# Autodesk Inventor assembly: XY Joint-Unit [A]
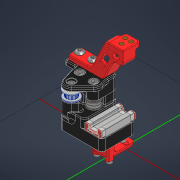
[picture p0: Inventor's stored thumbnail of the model, 180x180]
Saved by Autodesk Inventor 2022.2 (Build 262287010, 287A)
## iProperties
Created: 2022-03-15
Part Number: XY Joint-Unit [A]
Document SubType Name: Assembly
Designer: sleib
Author: sleib
## Documents named in this file (15)
- C:\Users\sleib\Projekte\Voron-2\CAD\Inventor\XY Joint-Unit [A].iam
- C:\Users\sleib\Projekte\Voron-2\CAD\Inventor\MGN9H Carriage.ipt
- C:\Users\sleib\Projekte\Voron-2\CAD\Inventor\M3x16 SHCS.ipt
- C:\Users\sleib\Projekte\Voron-2\CAD\Inventor\M3x30 SHCS.ipt
- C:\Users\sleib\Projekte\Voron-2\CAD\Inventor\XY Endstop Mount (Omron).ipt
- C:\Users\sleib\Projekte\Voron-2\CAD\Inventor\M5x40 SHCS.ipt
- C:\Users\sleib\Projekte\Voron-2\CAD\Inventor\GT2 20T Idler (6mm).ipt
- C:\Users\sleib\Projekte\Voron-2\CAD\Inventor\M5 Hexnut.ipt
- C:\Users\sleib\Projekte\Voron-2\CAD\Inventor\M5 Spacer (1mm).ipt
- C:\Users\sleib\Projekte\Voron-2\CAD\Inventor\Bearing F695-ZZ.ipt
- C:\Users\sleib\Projekte\Voron-2\CAD\Inventor\Chain Standoff (3-Hole).ipt
- C:\Users\sleib\Projekte\Voron-2\CAD\Inventor\M5x16 BHCS.ipt
- C:\Users\sleib\Projekte\Voron-2\CAD\Inventor\M5x30 BHCS.ipt
- C:\Users\sleib\Projekte\Voron-2\CAD\Inventor\XY Joint MGN12H [A].ipt
- C:\Users\sleib\Projekte\Voron-2\CAD\Inventor\M3 Threaded Insert.ipt
## Components (26 placed, 14 different names)
1. XY Joint MGN12H [A]:1 — Passend:50, Passend:51, Passend:52, Passend:53, Passend:54, Passend:55, Passend:56, Passend:57, Winkel:1, Winkel:2, Winkel:3, Passend:58, Passend:59, Passend:60, Passend:61, Passend:62, Passend:63, Passend:64, Passend:65, Passend:66, Passend:67, Passend:68, Passend:69, Passend:70, Passend:71, Passend:72, Passend:73, Passend:75, Passend:76, Passend:78, Passend:80, Passend:81, Passend:83, Passend:84
2. MGN9H Carriage:1 — Passend:10, Passend:11, Passend:12, Passend:13, Passend:69
3. XY Endstop Mount (Omron):1 — Passend:17, Passend:18, Passend:20, Passend:21, Passend:68
4. GT2 20T Idler (6mm):1 — Passend:23, Passend:83
5. Bearing F695-ZZ:1 — Passend:37, Passend:40, Passend:41
6. Bearing F695-ZZ:2 — Passend:38, Passend:41, Passend:42
7. M3x16 SHCS:1 — Passend:10, Passend:65, Passend:71
8. M3x16 SHCS:2 — Passend:11, Passend:64, Passend:70
9. M3x30 SHCS:1 — Passend:12, Passend:18, Passend:21, Passend:67
10. M3x30 SHCS:2 — Passend:13, Passend:17, Passend:20, Passend:66
11. M5x40 SHCS:1 — Passend:23, Passend:81, Passend:84
12. M5x40 SHCS:2 — Passend:36, Passend:37, Passend:38, Passend:39, Passend:74, Passend:76
13. M5x40 SHCS:3 — Passend:79, Passend:80
14. M5x40 SHCS:4 — Passend:77, Passend:78
15. M5 Hexnut:1 — Passend:50, Winkel:2, Passend:60, Passend:79
16. M5 Hexnut:2 — Passend:51, Winkel:1, Passend:58, Passend:74
17. M5 Hexnut:3 — Passend:52, Winkel:3, Passend:59, Passend:77
18. M5 Spacer (1mm):1 — Passend:36, Passend:40
19. M5 Spacer (1mm):2 — Passend:39, Passend:42, Passend:75
20. Chain Standoff (3-Hole):1 — Passend:46, Passend:47, Passend:48, Passend:49, Passend:63, Passend:85, Passend:86, Passend:87, Fluchtend:1, Fluchtend:2, Fluchtend:3
21. M5x16 BHCS:1 — Passend:46, Passend:48, Passend:61
22. M5x16 BHCS:2 — Passend:47, Passend:49, Passend:62
23. M5x30 BHCS:1 — Passend:72, Passend:73
24. M3 Threaded Insert:1 — Passend:86, Fluchtend:1
25. M3 Threaded Insert:2 — Passend:87, Fluchtend:2
26. M3 Threaded Insert:3 — Passend:85, Fluchtend:3
## Relationships (63: Mate 57, Angle 3, Flush 3)
- Passend:10 [Mate]: MGN9H Carriage:1 ↔ M3x16 SHCS:1
- Passend:11 [Mate]: MGN9H Carriage:1 ↔ M3x16 SHCS:2
- Passend:12 [Mate]: MGN9H Carriage:1 ↔ M3x30 SHCS:1
- Passend:13 [Mate]: MGN9H Carriage:1 ↔ M3x30 SHCS:2
- Passend:17 [Mate]: XY Endstop Mount (Omron):1 ↔ M3x30 SHCS:2
- Passend:18 [Mate]: XY Endstop Mount (Omron):1 ↔ M3x30 SHCS:1
- Passend:20 [Mate]: XY Endstop Mount (Omron):1 ↔ M3x30 SHCS:2
- Passend:21 [Mate]: XY Endstop Mount (Omron):1 ↔ M3x30 SHCS:1
- Passend:23 [Mate]: GT2 20T Idler (6mm):1 ↔ M5x40 SHCS:1
- Passend:36 [Mate]: M5x40 SHCS:2 ↔ M5 Spacer (1mm):1
- Passend:37 [Mate]: Bearing F695-ZZ:1 ↔ M5x40 SHCS:2
- Passend:38 [Mate]: Bearing F695-ZZ:2 ↔ M5x40 SHCS:2
- Passend:39 [Mate]: M5x40 SHCS:2 ↔ M5 Spacer (1mm):2
- Passend:40 [Mate]: Bearing F695-ZZ:1 ↔ M5 Spacer (1mm):1
- Passend:41 [Mate]: Bearing F695-ZZ:1 ↔ Bearing F695-ZZ:2
- Passend:42 [Mate]: Bearing F695-ZZ:2 ↔ M5 Spacer (1mm):2
- Passend:46 [Mate]: Chain Standoff (3-Hole):1 ↔ M5x16 BHCS:1
- Passend:47 [Mate]: Chain Standoff (3-Hole):1 ↔ M5x16 BHCS:2
- Passend:48 [Mate]: Chain Standoff (3-Hole):1 ↔ M5x16 BHCS:1
- Passend:49 [Mate]: Chain Standoff (3-Hole):1 ↔ M5x16 BHCS:2
- Passend:50 [Mate]: XY Joint MGN12H [A]:1 ↔ M5 Hexnut:1
- Passend:51 [Mate]: XY Joint MGN12H [A]:1 ↔ M5 Hexnut:2
- Passend:52 [Mate]: XY Joint MGN12H [A]:1 ↔ M5 Hexnut:3
- Passend:53 [Mate]: XY Joint MGN12H [A]:1
- Passend:54 [Mate]: XY Joint MGN12H [A]:1
- Passend:55 [Mate]: XY Joint MGN12H [A]:1
- Passend:56 [Mate] (7.5 mm): XY Joint MGN12H [A]:1
- Passend:57 [Mate] (7.5 mm): XY Joint MGN12H [A]:1
- Winkel:1 [Angle] (0 deg): XY Joint MGN12H [A]:1 ↔ M5 Hexnut:2
- Winkel:2 [Angle] (0 deg): XY Joint MGN12H [A]:1 ↔ M5 Hexnut:1
- Winkel:3 [Angle] (0 deg): XY Joint MGN12H [A]:1 ↔ M5 Hexnut:3
- Passend:58 [Mate]: XY Joint MGN12H [A]:1 ↔ M5 Hexnut:2
- Passend:59 [Mate]: XY Joint MGN12H [A]:1 ↔ M5 Hexnut:3
- Passend:60 [Mate]: XY Joint MGN12H [A]:1 ↔ M5 Hexnut:1
- Passend:61 [Mate]: XY Joint MGN12H [A]:1 ↔ M5x16 BHCS:1
- Passend:62 [Mate]: XY Joint MGN12H [A]:1 ↔ M5x16 BHCS:2
- Passend:63 [Mate]: XY Joint MGN12H [A]:1 ↔ Chain Standoff (3-Hole):1
- Passend:64 [Mate]: XY Joint MGN12H [A]:1 ↔ M3x16 SHCS:2
- Passend:65 [Mate]: XY Joint MGN12H [A]:1 ↔ M3x16 SHCS:1
- Passend:66 [Mate]: XY Joint MGN12H [A]:1 ↔ M3x30 SHCS:2
- Passend:67 [Mate]: XY Joint MGN12H [A]:1 ↔ M3x30 SHCS:1
- Passend:68 [Mate]: XY Joint MGN12H [A]:1 ↔ XY Endstop Mount (Omron):1
- Passend:69 [Mate]: XY Joint MGN12H [A]:1 ↔ MGN9H Carriage:1
- Passend:70 [Mate]: XY Joint MGN12H [A]:1 ↔ M3x16 SHCS:2
- Passend:71 [Mate]: XY Joint MGN12H [A]:1 ↔ M3x16 SHCS:1
- Passend:72 [Mate]: XY Joint MGN12H [A]:1 ↔ M5x30 BHCS:1
- Passend:73 [Mate]: XY Joint MGN12H [A]:1 ↔ M5x30 BHCS:1
- Passend:74 [Mate]: M5x40 SHCS:2 ↔ M5 Hexnut:2
- Passend:75 [Mate]: XY Joint MGN12H [A]:1 ↔ M5 Spacer (1mm):2
- Passend:76 [Mate]: XY Joint MGN12H [A]:1 ↔ M5x40 SHCS:2
- Passend:77 [Mate]: M5x40 SHCS:4 ↔ M5 Hexnut:3
- Passend:78 [Mate]: XY Joint MGN12H [A]:1 ↔ M5x40 SHCS:4
- Passend:79 [Mate]: M5x40 SHCS:3 ↔ M5 Hexnut:1
- Passend:80 [Mate]: XY Joint MGN12H [A]:1 ↔ M5x40 SHCS:3
- Passend:81 [Mate]: XY Joint MGN12H [A]:1 ↔ M5x40 SHCS:1
- Passend:83 [Mate]: XY Joint MGN12H [A]:1 ↔ GT2 20T Idler (6mm):1
- Passend:84 [Mate]: XY Joint MGN12H [A]:1 ↔ M5x40 SHCS:1
- Passend:85 [Mate]: Chain Standoff (3-Hole):1 ↔ M3 Threaded Insert:3
- Passend:86 [Mate]: Chain Standoff (3-Hole):1 ↔ M3 Threaded Insert:1
- Passend:87 [Mate]: Chain Standoff (3-Hole):1 ↔ M3 Threaded Insert:2
- Fluchtend:1 [Flush]: Chain Standoff (3-Hole):1 ↔ M3 Threaded Insert:1
- Fluchtend:2 [Flush]: Chain Standoff (3-Hole):1 ↔ M3 Threaded Insert:2
- Fluchtend:3 [Flush]: Chain Standoff (3-Hole):1 ↔ M3 Threaded Insert:3
